(part 1 of 2)
# Autodesk Inventor assembly: SAR340
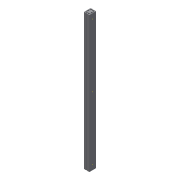
[picture p0: Inventor's stored thumbnail of the model, 180x180]
Saved by Autodesk Inventor 2020 (Build 240168000, 168)
## iProperties
Created: 2019-11-23
Part Number: SAR340
Catalog Web Link: www.cadenas.de
Description: SAR3-Slide Rails - Aluminum Alloy - Three-Step Slide Rails
Vendor: MISUMI
Document SubType Name: Assembly
Designer: psadmin
Manufacturer: MISUMI
Category: PARTsolutions
Company: MISUMI
PSOL_IDENT_0: {$CADENAS_DATA\23d-libs\misumi\metric\07_slide_rails\sar3_asmtab.prj},168 {VTYP=3D},{STYP=ASSTAB},{N
PSOL_IDENT_1: B=SAR340},{LINA=SAR340},{NN=SAR3},{DATE=09.09.2019 15:26:52},{GEOMDATE=01.03.2017 00:48:28},{VERSION=
PSOL_IDENT_2: },{LINEID=10},{WBVAR=NO},{WBNUMERIC=NO}  {NB=SAR340},{LINA=SAR340},{KT=DUMMY},{PN=SAR340},{TP=SAR3},
PSOL_IDENT_3: {TYPE=SAR3},{MAT1=Aluminum Alloy},{ST1=Clear Anodizing},{MAT2=Aluminum Alloy},{ST2=Clear Anodizing},
PSOL_IDENT_4: {MAT3=Steel},{NO=40},{RL=400},{TD=460},{A=185},{B=370},{C=185},{D=370},{RLO=147},{PPATH=sar3_series\
PSOL_IDENT_5: \sar3_templ.prj}
NN: SAR3
NT: Slide Rails - Aluminum Alloy - Three-Step Slide Rails
NB: SAR340
NBSYN: $PN.
LINA: SAR340
PN: SAR340
TP: SAR3
MAT1: Aluminum Alloy
ST1: Clear Anodizing
MAT2: Aluminum Alloy
ST2: Clear Anodizing
MAT3: Steel
NO: 40
RL: 400
TD: 460
A: 185
B: 370
C: 185
D: 370
RLO: 147
SUPPLIER: MISUMI
ARTICLENO: SAR340
BOMINFO: SAR340
CREATOR: CADENAS GmbH
Title: SAR340
Author: Cadenas PARTsolutions
Comments: Slide Rails - Aluminum Alloy - Three-Step Slide Rails
## Documents named in this file (4)
- C:\FTC\FTC8863CAD\Misumi\SAR340\SAR340.iam
- C:\FTC\FTC8863CAD\Misumi\SAR340\SAR340-40_r.ipt
- C:\FTC\FTC8863CAD\Misumi\SAR340\SAR340-40_b.ipt
- C:\FTC\FTC8863CAD\Misumi\SAR340\SAR3_ba.ipt
## Components (151 placed, 3 different names)
1. SAR340-40_r:1 — to_body_Z@1 <-> to_rail_Z@2, to_body_YZ@1 <-> to_rail_YZ@2, to_body2_Z@1 <-> to_rail_Z@3, to_body2_YZ@1 <-> to_rail_YZ@3, to_ball1_1_XY@1 <-> to_rail_XY@4, to_ball1_1_Z@1 <-> to_rail_Z@4, to_ball1_1_YZ@1 <-> to_rail_YZ@4, to_ball1_2_XY@1 <-> to_rail_XY@5, to_ball1_2_Z@1 <-> to_rail_Z@5, to_ball1_2_YZ@1 <-> to_rail_YZ@5, to_ball1_3_XY@1 <-> to_rail_XY@6, to_ball1_3_Z@1 <-> to_rail_Z@6, to_ball1_3_YZ@1 <-> to_rail_YZ@6, to_ball1_4_XY@1 <-> to_rail_XY@7, to_ball1_4_Z@1 <-> to_rail_Z@7, to_ball1_4_YZ@1 <-> to_rail_YZ@7, to_ball1_5_XY@1 <-> to_rail_XY@8, to_ball1_5_Z@1 <-> to_rail_Z@8, to_ball1_5_YZ@1 <-> to_rail_YZ@8, to_ball1_6_XY@1 <-> to_rail_XY@9, to_ball1_6_Z@1 <-> to_rail_Z@9, to_ball1_6_YZ@1 <-> to_rail_YZ@9, to_ball1_7_XY@1 <-> to_rail_XY@10, to_ball1_7_Z@1 <-> to_rail_Z@10, to_ball1_7_YZ@1 <-> to_rail_YZ@10, to_ball1_8_XY@1 <-> to_rail_XY@11, to_ball1_8_Z@1 <-> to_rail_Z@11, to_ball1_8_YZ@1 <-> to_rail_YZ@11, to_ball1_9_XY@1 <-> to_rail_XY@12, to_ball1_9_Z@1 <-> to_rail_Z@12, to_ball1_9_YZ@1 <-> to_rail_YZ@12, to_ball1_10_XY@1 <-> to_rail_XY@13, to_ball1_10_Z@1 <-> to_rail_Z@13, to_ball1_10_YZ@1 <-> to_rail_YZ@13, to_ball1_11_XY@1 <-> to_rail_XY@14, to_ball1_11_Z@1 <-> to_rail_Z@14, to_ball1_11_YZ@1 <-> to_rail_YZ@14, to_ball1_12_XY@1 <-> to_rail_XY@15, to_ball1_12_Z@1 <-> to_rail_Z@15, to_ball1_12_YZ@1 <-> to_rail_YZ@15, to_ball1_13_XY@1 <-> to_rail_XY@16, to_ball1_13_Z@1 <-> to_rail_Z@16, to_ball1_13_YZ@1 <-> to_rail_YZ@16, to_ball1_14_XY@1 <-> to_rail_XY@17, to_ball1_14_Z@1 <-> to_rail_Z@17, to_ball1_14_YZ@1 <-> to_rail_YZ@17, to_ball1_15_XY@1 <-> to_rail_XY@18, to_ball1_15_Z@1 <-> to_rail_Z@18, to_ball1_15_YZ@1 <-> to_rail_YZ@18, to_ball1_16_XY@1 <-> to_rail_XY@19, to_ball1_16_Z@1 <-> to_rail_Z@19, to_ball1_16_YZ@1 <-> to_rail_YZ@19, to_ball1_17_XY@1 <-> to_rail_XY@20, to_ball1_17_Z@1 <-> to_rail_Z@20, to_ball1_17_YZ@1 <-> to_rail_YZ@20, to_ball1_18_XY@1 <-> to_rail_XY@21, to_ball1_18_Z@1 <-> to_rail_Z@21, to_ball1_18_YZ@1 <-> to_rail_YZ@21, to_ball1_19_XY@1 <-> to_rail_XY@22, to_ball1_19_Z@1 <-> to_rail_Z@22, to_ball1_19_YZ@1 <-> to_rail_YZ@22, to_ball1_20_XY@1 <-> to_rail_XY@23, to_ball1_20_Z@1 <-> to_rail_Z@23, to_ball1_20_YZ@1 <-> to_rail_YZ@23, to_ball1_21_XY@1 <-> to_rail_XY@24, to_ball1_21_Z@1 <-> to_rail_Z@24, to_ball1_21_YZ@1 <-> to_rail_YZ@24, to_ball1_22_XY@1 <-> to_rail_XY@25, to_ball1_22_Z@1 <-> to_rail_Z@25, to_ball1_22_YZ@1 <-> to_rail_YZ@25, to_ball1_23_XY@1 <-> to_rail_XY@26, to_ball1_23_Z@1 <-> to_rail_Z@26, to_ball1_23_YZ@1 <-> to_rail_YZ@26, to_ball1_24_XY@1 <-> to_rail_XY@27, to_ball1_24_Z@1 <-> to_rail_Z@27, to_ball1_24_YZ@1 <-> to_rail_YZ@27, to_ball1_25_XY@1 <-> to_rail_XY@28, to_ball1_25_Z@1 <-> to_rail_Z@28, to_ball1_25_YZ@1 <-> to_rail_YZ@28, to_ball1_26_XY@1 <-> to_rail_XY@29, to_ball1_26_Z@1 <-> to_rail_Z@29, to_ball1_26_YZ@1 <-> to_rail_YZ@29, to_ball1_27_XY@1 <-> to_rail_XY@30, to_ball1_27_Z@1 <-> to_rail_Z@30, to_ball1_27_YZ@1 <-> to_rail_YZ@30, to_ball1_28_XY@1 <-> to_rail_XY@31, to_ball1_28_Z@1 <-> to_rail_Z@31, to_ball1_28_YZ@1 <-> to_rail_YZ@31, to_ball1_29_XY@1 <-> to_rail_XY@32, to_ball1_29_Z@1 <-> to_rail_Z@32, to_ball1_29_YZ@1 <-> to_rail_YZ@32, to_ball1_30_XY@1 <-> to_rail_XY@33, to_ball1_30_Z@1 <-> to_rail_Z@33, to_ball1_30_YZ@1 <-> to_rail_YZ@33, to_ball1_31_XY@1 <-> to_rail_XY@34, to_ball1_31_Z@1 <-> to_rail_Z@34, to_ball1_31_YZ@1 <-> to_rail_YZ@34, to_ball1_32_XY@1 <-> to_rail_XY@35, to_ball1_32_Z@1 <-> to_rail_Z@35, to_ball1_32_YZ@1 <-> to_rail_YZ@35, to_ball1_33_XY@1 <-> to_rail_XY@36, to_ball1_33_Z@1 <-> to_rail_Z@36, to_ball1_33_YZ@1 <-> to_rail_YZ@36, to_ball1_34_XY@1 <-> to_rail_XY@37, to_ball1_34_Z@1 <-> to_rail_Z@37, to_ball1_34_YZ@1 <-> to_rail_YZ@37, to_ball1_35_XY@1 <-> to_rail_XY@38, to_ball1_35_Z@1 <-> to_rail_Z@38, to_ball1_35_YZ@1 <-> to_rail_YZ@38, to_ball1_36_XY@1 <-> to_rail_XY@39, to_ball1_36_Z@1 <-> to_rail_Z@39, to_ball1_36_YZ@1 <-> to_rail_YZ@39, to_ball1_37_XY@1 <-> to_rail_XY@40, to_ball1_37_Z@1 <-> to_rail_Z@40, to_ball1_37_YZ@1 <-> to_rail_YZ@40, to_ball2_1_XY@1 <-> to_rail_XY@41, to_ball2_1_Z@1 <-> to_rail_Z@41, to_ball2_1_YZ@1 <-> to_rail_YZ@41, to_ball2_2_XY@1 <-> to_rail_XY@42, to_ball2_2_Z@1 <-> to_rail_Z@42, to_ball2_2_YZ@1 <-> to_rail_YZ@42, to_ball2_3_XY@1 <-> to_rail_XY@43, to_ball2_3_Z@1 <-> to_rail_Z@43, to_ball2_3_YZ@1 <-> to_rail_YZ@43, to_ball2_4_XY@1 <-> to_rail_XY@44, to_ball2_4_Z@1 <-> to_rail_Z@44, to_ball2_4_YZ@1 <-> to_rail_YZ@44, to_ball2_5_XY@1 <-> to_rail_XY@45, to_ball2_5_Z@1 <-> to_rail_Z@45, to_ball2_5_YZ@1 <-> to_rail_YZ@45, to_ball2_6_XY@1 <-> to_rail_XY@46, to_ball2_6_Z@1 <-> to_rail_Z@46, to_ball2_6_YZ@1 <-> to_rail_YZ@46, to_ball2_7_XY@1 <-> to_rail_XY@47, to_ball2_7_Z@1 <-> to_rail_Z@47, to_ball2_7_YZ@1 <-> to_rail_YZ@47, to_ball2_8_XY@1 <-> to_rail_XY@48, to_ball2_8_Z@1 <-> to_rail_Z@48, to_ball2_8_YZ@1 <-> to_rail_YZ@48, to_ball2_9_XY@1 <-> to_rail_XY@49, to_ball2_9_Z@1 <-> to_rail_Z@49, to_ball2_9_YZ@1 <-> to_rail_YZ@49, to_ball2_10_XY@1 <-> to_rail_XY@50, to_ball2_10_Z@1 <-> to_rail_Z@50, to_ball2_10_YZ@1 <-> to_rail_YZ@50, to_ball2_11_XY@1 <-> to_rail_XY@51, to_ball2_11_Z@1 <-> to_rail_Z@51, to_ball2_11_YZ@1 <-> to_rail_YZ@51, to_ball2_12_XY@1 <-> to_rail_XY@52, to_ball2_12_Z@1 <-> to_rail_Z@52, to_ball2_12_YZ@1 <-> to_rail_YZ@52, to_ball2_13_XY@1 <-> to_rail_XY@53, to_ball2_13_Z@1 <-> to_rail_Z@53, to_ball2_13_YZ@1 <-> to_rail_YZ@53, to_ball2_14_XY@1 <-> to_rail_XY@54, to_ball2_14_Z@1 <-> to_rail_Z@54, to_ball2_14_YZ@1 <-> to_rail_YZ@54, to_ball2_15_XY@1 <-> to_rail_XY@55, to_ball2_15_Z@1 <-> to_rail_Z@55, to_ball2_15_YZ@1 <-> to_rail_YZ@55, to_ball2_16_XY@1 <-> to_rail_XY@56, to_ball2_16_Z@1 <-> to_rail_Z@56, to_ball2_16_YZ@1 <-> to_rail_YZ@56, to_ball2_17_XY@1 <-> to_rail_XY@57, to_ball2_17_Z@1 <-> to_rail_Z@57, to_ball2_17_YZ@1 <-> to_rail_YZ@57, to_ball2_18_XY@1 <-> to_rail_XY@58, to_ball2_18_Z@1 <-> to_rail_Z@58, to_ball2_18_YZ@1 <-> to_rail_YZ@58, to_ball2_19_XY@1 <-> to_rail_XY@59, to_ball2_19_Z@1 <-> to_rail_Z@59, to_ball2_19_YZ@1 <-> to_rail_YZ@59, to_ball2_20_XY@1 <-> to_rail_XY@60, to_ball2_20_Z@1 <-> to_rail_Z@60, to_ball2_20_YZ@1 <-> to_rail_YZ@60, to_ball2_21_XY@1 <-> to_rail_XY@61, to_ball2_21_Z@1 <-> to_rail_Z@61, to_ball2_21_YZ@1 <-> to_rail_YZ@61, to_ball2_22_XY@1 <-> to_rail_XY@62, to_ball2_22_Z@1 <-> to_rail_Z@62, to_ball2_22_YZ@1 <-> to_rail_YZ@62, to_ball2_23_XY@1 <-> to_rail_XY@63, to_ball2_23_Z@1 <-> to_rail_Z@63, to_ball2_23_YZ@1 <-> to_rail_YZ@63, to_ball2_24_XY@1 <-> to_rail_XY@64, to_ball2_24_Z@1 <-> to_rail_Z@64, to_ball2_24_YZ@1 <-> to_rail_YZ@64, to_ball2_25_XY@1 <-> to_rail_XY@65, to_ball2_25_Z@1 <-> to_rail_Z@65, to_ball2_25_YZ@1 <-> to_rail_YZ@65, to_ball2_26_XY@1 <-> to_rail_XY@66, to_ball2_26_Z@1 <-> to_rail_Z@66, to_ball2_26_YZ@1 <-> to_rail_YZ@66, to_ball2_27_XY@1 <-> to_rail_XY@67, to_ball2_27_Z@1 <-> to_rail_Z@67, to_ball2_27_YZ@1 <-> to_rail_YZ@67, to_ball2_28_XY@1 <-> to_rail_XY@68, to_ball2_28_Z@1 <-> to_rail_Z@68, to_ball2_28_YZ@1 <-> to_rail_YZ@68, to_ball2_29_XY@1 <-> to_rail_XY@69, to_ball2_29_Z@1 <-> to_rail_Z@69, to_ball2_29_YZ@1 <-> to_rail_YZ@69, to_ball2_30_XY@1 <-> to_rail_XY@70, to_ball2_30_Z@1 <-> to_rail_Z@70, to_ball2_30_YZ@1 <-> to_rail_YZ@70, to_ball2_31_XY@1 <-> to_rail_XY@71, to_ball2_31_Z@1 <-> to_rail_Z@71, to_ball2_31_YZ@1 <-> to_rail_YZ@71, to_ball2_32_XY@1 <-> to_rail_XY@72, to_ball2_32_Z@1 <-> to_rail_Z@72, to_ball2_32_YZ@1 <-> to_rail_YZ@72, to_ball2_33_XY@1 <-> to_rail_XY@73, to_ball2_33_Z@1 <-> to_rail_Z@73, to_ball2_33_YZ@1 <-> to_rail_YZ@73, to_ball2_34_XY@1 <-> to_rail_XY@74, to_ball2_34_Z@1 <-> to_rail_Z@74, to_ball2_34_YZ@1 <-> to_rail_YZ@74, to_ball2_35_XY@1 <-> to_rail_XY@75, to_ball2_35_Z@1 <-> to_rail_Z@75, to_ball2_35_YZ@1 <-> to_rail_YZ@75, to_ball2_36_XY@1 <-> to_rail_XY@76, to_ball2_36_Z@1 <-> to_rail_Z@76, to_ball2_36_YZ@1 <-> to_rail_YZ@76, to_ball2_37_XY@1 <-> to_rail_XY@77, to_ball2_37_Z@1 <-> to_rail_Z@77, to_ball2_37_YZ@1 <-> to_rail_YZ@77, to_ball3_1_XY@1 <-> to_rail_XY@78, to_ball3_1_Z@1 <-> to_rail_Z@78, to_ball3_1_YZ@1 <-> to_rail_YZ@78, to_ball3_2_XY@1 <-> to_rail_XY@79, to_ball3_2_Z@1 <-> to_rail_Z@79, to_ball3_2_YZ@1 <-> to_rail_YZ@79, to_ball3_3_XY@1 <-> to_rail_XY@80, to_ball3_3_Z@1 <-> to_rail_Z@80, to_ball3_3_YZ@1 <-> to_rail_YZ@80, to_ball3_4_XY@1 <-> to_rail_XY@81, to_ball3_4_Z@1 <-> to_rail_Z@81, to_ball3_4_YZ@1 <-> to_rail_YZ@81, to_ball3_5_XY@1 <-> to_rail_XY@82, to_ball3_5_Z@1 <-> to_rail_Z@82, to_ball3_5_YZ@1 <-> to_rail_YZ@82, to_ball3_6_XY@1 <-> to_rail_XY@83, to_ball3_6_Z@1 <-> to_rail_Z@83, to_ball3_6_YZ@1 <-> to_rail_YZ@83, to_ball3_7_XY@1 <-> to_rail_XY@84, to_ball3_7_Z@1 <-> to_rail_Z@84, to_ball3_7_YZ@1 <-> to_rail_YZ@84, to_ball3_8_XY@1 <-> to_rail_XY@85, to_ball3_8_Z@1 <-> to_rail_Z@85, to_ball3_8_YZ@1 <-> to_rail_YZ@85, to_ball3_9_XY@1 <-> to_rail_XY@86, to_ball3_9_Z@1 <-> to_rail_Z@86, to_ball3_9_YZ@1 <-> to_rail_YZ@86, to_ball3_10_XY@1 <-> to_rail_XY@87, to_ball3_10_Z@1 <-> to_rail_Z@87, to_ball3_10_YZ@1 <-> to_rail_YZ@87, to_ball3_11_XY@1 <-> to_rail_XY@88, to_ball3_11_Z@1 <-> to_rail_Z@88, to_ball3_11_YZ@1 <-> to_rail_YZ@88, to_ball3_12_XY@1 <-> to_rail_XY@89, to_ball3_12_Z@1 <-> to_rail_Z@89, to_ball3_12_YZ@1 <-> to_rail_YZ@89, to_ball3_13_XY@1 <-> to_rail_XY@90, to_ball3_13_Z@1 <-> to_rail_Z@90, to_ball3_13_YZ@1 <-> to_rail_YZ@90, to_ball3_14_XY@1 <-> to_rail_XY@91, to_ball3_14_Z@1 <-> to_rail_Z@91, to_ball3_14_YZ@1 <-> to_rail_YZ@91, to_ball3_15_XY@1 <-> to_rail_XY@92, to_ball3_15_Z@1 <-> to_rail_Z@92, to_ball3_15_YZ@1 <-> to_rail_YZ@92, to_ball3_16_XY@1 <-> to_rail_XY@93, to_ball3_16_Z@1 <-> to_rail_Z@93, to_ball3_16_YZ@1 <-> to_rail_YZ@93, to_ball3_17_XY@1 <-> to_rail_XY@94, to_ball3_17_Z@1 <-> to_rail_Z@94, to_ball3_17_YZ@1 <-> to_rail_YZ@94, to_ball3_18_XY@1 <-> to_rail_XY@95, to_ball3_18_Z@1 <-> to_rail_Z@95, to_ball3_18_YZ@1 <-> to_rail_YZ@95, to_ball3_19_XY@1 <-> to_rail_XY@96, to_ball3_19_Z@1 <-> to_rail_Z@96, to_ball3_19_YZ@1 <-> to_rail_YZ@96, to_ball3_20_XY@1 <-> to_rail_XY@97, to_ball3_20_Z@1 <-> to_rail_Z@97, to_ball3_20_YZ@1 <-> to_rail_YZ@97, to_ball3_21_XY@1 <-> to_rail_XY@98, to_ball3_21_Z@1 <-> to_rail_Z@98, to_ball3_21_YZ@1 <-> to_rail_YZ@98, to_ball3_22_XY@1 <-> to_rail_XY@99, to_ball3_22_Z@1 <-> to_rail_Z@99, to_ball3_22_YZ@1 <-> to_rail_YZ@99, to_ball3_23_XY@1 <-> to_rail_XY@100, to_ball3_23_Z@1 <-> to_rail_Z@100, to_ball3_23_YZ@1 <-> to_rail_YZ@100, to_ball3_24_XY@1 <-> to_rail_XY@101, to_ball3_24_Z@1 <-> to_rail_Z@101, to_ball3_24_YZ@1 <-> to_rail_YZ@101, to_ball3_25_XY@1 <-> to_rail_XY@102, to_ball3_25_Z@1 <-> to_rail_Z@102, to_ball3_25_YZ@1 <-> to_rail_YZ@102, to_ball3_26_XY@1 <-> to_rail_XY@103, to_ball3_26_Z@1 <-> to_rail_Z@103, to_ball3_26_YZ@1 <-> to_rail_YZ@103, to_ball3_27_XY@1 <-> to_rail_XY@104, to_ball3_27_Z@1 <-> to_rail_Z@104, to_ball3_27_YZ@1 <-> to_rail_YZ@104, to_ball3_28_XY@1 <-> to_rail_XY@105, to_ball3_28_Z@1 <-> to_rail_Z@105, to_ball3_28_YZ@1 <-> to_rail_YZ@105, to_ball3_29_XY@1 <-> to_rail_XY@106, to_ball3_29_Z@1 <-> to_rail_Z@106, to_ball3_29_YZ@1 <-> to_rail_YZ@106, to_ball3_30_XY@1 <-> to_rail_XY@107, to_ball3_30_Z@1 <-> to_rail_Z@107, to_ball3_30_YZ@1 <-> to_rail_YZ@107, to_ball3_31_XY@1 <-> to_rail_XY@108, to_ball3_31_Z@1 <-> to_rail_Z@108, to_ball3_31_YZ@1 <-> to_rail_YZ@108, to_ball3_32_XY@1 <-> to_rail_XY@109, to_ball3_32_Z@1 <-> to_rail_Z@109, to_ball3_32_YZ@1 <-> to_rail_YZ@109, to_ball3_33_XY@1 <-> to_rail_XY@110, to_ball3_33_Z@1 <-> to_rail_Z@110, to_ball3_33_YZ@1 <-> to_rail_YZ@110, to_ball3_34_XY@1 <-> to_rail_XY@111, to_ball3_34_Z@1 <-> to_rail_Z@111, to_ball3_34_YZ@1 <-> to_rail_YZ@111, to_ball3_35_XY@1 <-> to_rail_XY@112, to_ball3_35_Z@1 <-> to_rail_Z@112, to_ball3_35_YZ@1 <-> to_rail_YZ@112, to_ball3_36_XY@1 <-> to_rail_XY@113, to_ball3_36_Z@1 <-> to_rail_Z@113, to_ball3_36_YZ@1 <-> to_rail_YZ@113, to_ball3_37_XY@1 <-> to_rail_XY@114, to_ball3_37_Z@1 <-> to_rail_Z@114, to_ball3_37_YZ@1 <-> to_rail_YZ@114, to_ball4_1_XY@1 <-> to_rail_XY@115, to_ball4_1_Z@1 <-> to_rail_Z@115, to_ball4_1_YZ@1 <-> to_rail_YZ@115, to_ball4_2_XY@1 <-> to_rail_XY@116, to_ball4_2_Z@1 <-> to_rail_Z@116, to_ball4_2_YZ@1 <-> to_rail_YZ@116, to_ball4_3_XY@1 <-> to_rail_XY@117, to_ball4_3_Z@1 <-> to_rail_Z@117, to_ball4_3_YZ@1 <-> to_rail_YZ@117, to_ball4_4_XY@1 <-> to_rail_XY@118, to_ball4_4_Z@1 <-> to_rail_Z@118, to_ball4_4_YZ@1 <-> to_rail_YZ@118, to_ball4_5_XY@1 <-> to_rail_XY@119, to_ball4_5_Z@1 <-> to_rail_Z@119, to_ball4_5_YZ@1 <-> to_rail_YZ@119, to_ball4_6_XY@1 <-> to_rail_XY@120, to_ball4_6_Z@1 <-> to_rail_Z@120, to_ball4_6_YZ@1 <-> to_rail_YZ@120, to_ball4_7_XY@1 <-> to_rail_XY@121, to_ball4_7_Z@1 <-> to_rail_Z@121, to_ball4_7_YZ@1 <-> to_rail_YZ@121, to_ball4_8_XY@1 <-> to_rail_XY@122, to_ball4_8_Z@1 <-> to_rail_Z@122, to_ball4_8_YZ@1 <-> to_rail_YZ@122, to_ball4_9_XY@1 <-> to_rail_XY@123, to_ball4_9_Z@1 <-> to_rail_Z@123, to_ball4_9_YZ@1 <-> to_rail_YZ@123, to_ball4_10_XY@1 <-> to_rail_XY@124, to_ball4_10_Z@1 <-> to_rail_Z@124, to_ball4_10_YZ@1 <-> to_rail_YZ@124, to_ball4_11_XY@1 <-> to_rail_XY@125, to_ball4_11_Z@1 <-> to_rail_Z@125, to_ball4_11_YZ@1 <-> to_rail_YZ@125, to_ball4_12_XY@1 <-> to_rail_XY@126, to_ball4_12_Z@1 <-> to_rail_Z@126, to_ball4_12_YZ@1 <-> to_rail_YZ@126, to_ball4_13_XY@1 <-> to_rail_XY@127, to_ball4_13_Z@1 <-> to_rail_Z@127, to_ball4_13_YZ@1 <-> to_rail_YZ@127, to_ball4_14_XY@1 <-> to_rail_XY@128, to_ball4_14_Z@1 <-> to_rail_Z@128, to_ball4_14_YZ@1 <-> to_rail_YZ@128, to_ball4_15_XY@1 <-> to_rail_XY@129, to_ball4_15_Z@1 <-> to_rail_Z@129, to_ball4_15_YZ@1 <-> to_rail_YZ@129, to_ball4_16_XY@1 <-> to_rail_XY@130, to_ball4_16_Z@1 <-> to_rail_Z@130, to_ball4_16_YZ@1 <-> to_rail_YZ@130, to_ball4_17_XY@1 <-> to_rail_XY@131, to_ball4_17_Z@1 <-> to_rail_Z@131, to_ball4_17_YZ@1 <-> to_rail_YZ@131, to_ball4_18_XY@1 <-> to_rail_XY@132, to_ball4_18_Z@1 <-> to_rail_Z@132, to_ball4_18_YZ@1 <-> to_rail_YZ@132, to_ball4_19_XY@1 <-> to_rail_XY@133, to_ball4_19_Z@1 <-> to_rail_Z@133, to_ball4_19_YZ@1 <-> to_rail_YZ@133, to_ball4_20_XY@1 <-> to_rail_XY@134, to_ball4_20_Z@1 <-> to_rail_Z@134, to_ball4_20_YZ@1 <-> to_rail_YZ@134, to_ball4_21_XY@1 <-> to_rail_XY@135, to_ball4_21_Z@1 <-> to_rail_Z@135, to_ball4_21_YZ@1 <-> to_rail_YZ@135, to_ball4_22_XY@1 <-> to_rail_XY@136, to_ball4_22_Z@1 <-> to_rail_Z@136, to_ball4_22_YZ@1 <-> to_rail_YZ@136, to_ball4_23_XY@1 <-> to_rail_XY@137, to_ball4_23_Z@1 <-> to_rail_Z@137, to_ball4_23_YZ@1 <-> to_rail_YZ@137, to_ball4_24_XY@1 <-> to_rail_XY@138, to_ball4_24_Z@1 <-> to_rail_Z@138, to_ball4_24_YZ@1 <-> to_rail_YZ@138, to_ball4_25_XY@1 <-> to_rail_XY@139, to_ball4_25_Z@1 <-> to_rail_Z@139, to_ball4_25_YZ@1 <-> to_rail_YZ@139, to_ball4_26_XY@1 <-> to_rail_XY@140, to_ball4_26_Z@1 <-> to_rail_Z@140, to_ball4_26_YZ@1 <-> to_rail_YZ@140, to_ball4_27_XY@1 <-> to_rail_XY@141, to_ball4_27_Z@1 <-> to_rail_Z@141, to_ball4_27_YZ@1 <-> to_rail_YZ@141, to_ball4_28_XY@1 <-> to_rail_XY@142, to_ball4_28_Z@1 <-> to_rail_Z@142, to_ball4_28_YZ@1 <-> to_rail_YZ@142, to_ball4_29_XY@1 <-> to_rail_XY@143, to_ball4_29_Z@1 <-> to_rail_Z@143, to_ball4_29_YZ@1 <-> to_rail_YZ@143, to_ball4_30_XY@1 <-> to_rail_XY@144, to_ball4_30_Z@1 <-> to_rail_Z@144, to_ball4_30_YZ@1 <-> to_rail_YZ@144, to_ball4_31_XY@1 <-> to_rail_XY@145, to_ball4_31_Z@1 <-> to_rail_Z@145, to_ball4_31_YZ@1 <-> to_rail_YZ@145, to_ball4_32_XY@1 <-> to_rail_XY@146, to_ball4_32_Z@1 <-> to_rail_Z@146, to_ball4_32_YZ@1 <-> to_rail_YZ@146, to_ball4_33_XY@1 <-> to_rail_XY@147, to_ball4_33_Z@1 <-> to_rail_Z@147, to_ball4_33_YZ@1 <-> to_rail_YZ@147, to_ball4_34_XY@1 <-> to_rail_XY@148, to_ball4_34_Z@1 <-> to_rail_Z@148, to_ball4_34_YZ@1 <-> to_rail_YZ@148, to_ball4_35_XY@1 <-> to_rail_XY@149, to_ball4_35_Z@1 <-> to_rail_Z@149, to_ball4_35_YZ@1 <-> to_rail_YZ@149, to_ball4_36_XY@1 <-> to_rail_XY@150, to_ball4_36_Z@1 <-> to_rail_Z@150, to_ball4_36_YZ@1 <-> to_rail_YZ@150, to_ball4_37_XY@1 <-> to_rail_XY@151, to_ball4_37_Z@1 <-> to_rail_Z@151, to_ball4_37_YZ@1 <-> to_rail_YZ@151
2. SAR340-40_b:1 — to_body_Z@1 <-> to_rail_Z@2, to_body_YZ@1 <-> to_rail_YZ@2, Mate:302, Mate:303, Mate:304
3. SAR340-40_b:2 — to_body2_Z@1 <-> to_rail_Z@3, to_body2_YZ@1 <-> to_rail_YZ@3, Mate:299, Mate:300, Mate:301
4. SAR3_ba:1 — to_ball1_1_XY@1 <-> to_rail_XY@4, to_ball1_1_Z@1 <-> to_rail_Z@4, to_ball1_1_YZ@1 <-> to_rail_YZ@4
5. SAR3_ba:2 — to_ball1_2_XY@1 <-> to_rail_XY@5, to_ball1_2_Z@1 <-> to_rail_Z@5, to_ball1_2_YZ@1 <-> to_rail_YZ@5
6. SAR3_ba:3 — to_ball1_3_XY@1 <-> to_rail_XY@6, to_ball1_3_Z@1 <-> to_rail_Z@6, to_ball1_3_YZ@1 <-> to_rail_YZ@6
7. SAR3_ba:4 — to_ball1_4_XY@1 <-> to_rail_XY@7, to_ball1_4_Z@1 <-> to_rail_Z@7, to_ball1_4_YZ@1 <-> to_rail_YZ@7
8. SAR3_ba:5 — to_ball1_5_XY@1 <-> to_rail_XY@8, to_ball1_5_Z@1 <-> to_rail_Z@8, to_ball1_5_YZ@1 <-> to_rail_YZ@8
9. SAR3_ba:6 — to_ball1_6_XY@1 <-> to_rail_XY@9, to_ball1_6_Z@1 <-> to_rail_Z@9, to_ball1_6_YZ@1 <-> to_rail_YZ@9
10. SAR3_ba:7 — to_ball1_7_XY@1 <-> to_rail_XY@10, to_ball1_7_Z@1 <-> to_rail_Z@10, to_ball1_7_YZ@1 <-> to_rail_YZ@10
11. SAR3_ba:8 — to_ball1_8_XY@1 <-> to_rail_XY@11, to_ball1_8_Z@1 <-> to_rail_Z@11, to_ball1_8_YZ@1 <-> to_rail_YZ@11
12. SAR3_ba:9 — to_ball1_9_XY@1 <-> to_rail_XY@12, to_ball1_9_Z@1 <-> to_rail_Z@12, to_ball1_9_YZ@1 <-> to_rail_YZ@12
13. SAR3_ba:10 — to_ball1_10_XY@1 <-> to_rail_XY@13, to_ball1_10_Z@1 <-> to_rail_Z@13, to_ball1_10_YZ@1 <-> to_rail_YZ@13
14. SAR3_ba:11 — to_ball1_11_XY@1 <-> to_rail_XY@14, to_ball1_11_Z@1 <-> to_rail_Z@14, to_ball1_11_YZ@1 <-> to_rail_YZ@14
15. SAR3_ba:12 — to_ball1_12_XY@1 <-> to_rail_XY@15, to_ball1_12_Z@1 <-> to_rail_Z@15, to_ball1_12_YZ@1 <-> to_rail_YZ@15
16. SAR3_ba:13 — to_ball1_13_XY@1 <-> to_rail_XY@16, to_ball1_13_Z@1 <-> to_rail_Z@16, to_ball1_13_YZ@1 <-> to_rail_YZ@16
17. SAR3_ba:14 — to_ball1_14_XY@1 <-> to_rail_XY@17, to_ball1_14_Z@1 <-> to_rail_Z@17, to_ball1_14_YZ@1 <-> to_rail_YZ@17
18. SAR3_ba:15 — to_ball1_15_XY@1 <-> to_rail_XY@18, to_ball1_15_Z@1 <-> to_rail_Z@18, to_ball1_15_YZ@1 <-> to_rail_YZ@18
19. SAR3_ba:16 — to_ball1_16_XY@1 <-> to_rail_XY@19, to_ball1_16_Z@1 <-> to_rail_Z@19, to_ball1_16_YZ@1 <-> to_rail_YZ@19
20. SAR3_ba:17 — to_ball1_17_XY@1 <-> to_rail_XY@20, to_ball1_17_Z@1 <-> to_rail_Z@20, to_ball1_17_YZ@1 <-> to_rail_YZ@20
21. SAR3_ba:18 — to_ball1_18_XY@1 <-> to_rail_XY@21, to_ball1_18_Z@1 <-> to_rail_Z@21, to_ball1_18_YZ@1 <-> to_rail_YZ@21
22. SAR3_ba:19 — to_ball1_19_XY@1 <-> to_rail_XY@22, to_ball1_19_Z@1 <-> to_rail_Z@22, to_ball1_19_YZ@1 <-> to_rail_YZ@22
23. SAR3_ba:20 — to_ball1_20_XY@1 <-> to_rail_XY@23, to_ball1_20_Z@1 <-> to_rail_Z@23, to_ball1_20_YZ@1 <-> to_rail_YZ@23
24. SAR3_ba:21 — to_ball1_21_XY@1 <-> to_rail_XY@24, to_ball1_21_Z@1 <-> to_rail_Z@24, to_ball1_21_YZ@1 <-> to_rail_YZ@24
25. SAR3_ba:22 — to_ball1_22_XY@1 <-> to_rail_XY@25, to_ball1_22_Z@1 <-> to_rail_Z@25, to_ball1_22_YZ@1 <-> to_rail_YZ@25
26. SAR3_ba:23 — to_ball1_23_XY@1 <-> to_rail_XY@26, to_ball1_23_Z@1 <-> to_rail_Z@26, to_ball1_23_YZ@1 <-> to_rail_YZ@26
27. SAR3_ba:24 — to_ball1_24_XY@1 <-> to_rail_XY@27, to_ball1_24_Z@1 <-> to_rail_Z@27, to_ball1_24_YZ@1 <-> to_rail_YZ@27
28. SAR3_ba:25 — to_ball1_25_XY@1 <-> to_rail_XY@28, to_ball1_25_Z@1 <-> to_rail_Z@28, to_ball1_25_YZ@1 <-> to_rail_YZ@28
29. SAR3_ba:26 — to_ball1_26_XY@1 <-> to_rail_XY@29, to_ball1_26_Z@1 <-> to_rail_Z@29, to_ball1_26_YZ@1 <-> to_rail_YZ@29
30. SAR3_ba:27 — to_ball1_27_XY@1 <-> to_rail_XY@30, to_ball1_27_Z@1 <-> to_rail_Z@30, to_ball1_27_YZ@1 <-> to_rail_YZ@30
31. SAR3_ba:28 — to_ball1_28_XY@1 <-> to_rail_XY@31, to_ball1_28_Z@1 <-> to_rail_Z@31, to_ball1_28_YZ@1 <-> to_rail_YZ@31
32. SAR3_ba:29 — to_ball1_29_XY@1 <-> to_rail_XY@32, to_ball1_29_Z@1 <-> to_rail_Z@32, to_ball1_29_YZ@1 <-> to_rail_YZ@32
33. SAR3_ba:30 — to_ball1_30_XY@1 <-> to_rail_XY@33, to_ball1_30_Z@1 <-> to_rail_Z@33, to_ball1_30_YZ@1 <-> to_rail_YZ@33
34. SAR3_ba:31 — to_ball1_31_XY@1 <-> to_rail_XY@34, to_ball1_31_Z@1 <-> to_rail_Z@34, to_ball1_31_YZ@1 <-> to_rail_YZ@34
35. SAR3_ba:32 — to_ball1_32_XY@1 <-> to_rail_XY@35, to_ball1_32_Z@1 <-> to_rail_Z@35, to_ball1_32_YZ@1 <-> to_rail_YZ@35
36. SAR3_ba:33 — to_ball1_33_XY@1 <-> to_rail_XY@36, to_ball1_33_Z@1 <-> to_rail_Z@36, to_ball1_33_YZ@1 <-> to_rail_YZ@36
37. SAR3_ba:34 — to_ball1_34_XY@1 <-> to_rail_XY@37, to_ball1_34_Z@1 <-> to_rail_Z@37, to_ball1_34_YZ@1 <-> to_rail_YZ@37
38. SAR3_ba:35 — to_ball1_35_XY@1 <-> to_rail_XY@38, to_ball1_35_Z@1 <-> to_rail_Z@38, to_ball1_35_YZ@1 <-> to_rail_YZ@38
39. SAR3_ba:36 — to_ball1_36_XY@1 <-> to_rail_XY@39, to_ball1_36_Z@1 <-> to_rail_Z@39, to_ball1_36_YZ@1 <-> to_rail_YZ@39
40. SAR3_ba:37 — to_ball1_37_XY@1 <-> to_rail_XY@40, to_ball1_37_Z@1 <-> to_rail_Z@40, to_ball1_37_YZ@1 <-> to_rail_YZ@40
41. SAR3_ba:38 — to_ball2_1_XY@1 <-> to_rail_XY@41, to_ball2_1_Z@1 <-> to_rail_Z@41, to_ball2_1_YZ@1 <-> to_rail_YZ@41
42. SAR3_ba:39 — to_ball2_2_XY@1 <-> to_rail_XY@42, to_ball2_2_Z@1 <-> to_rail_Z@42, to_ball2_2_YZ@1 <-> to_rail_YZ@42
43. SAR3_ba:40 — to_ball2_3_XY@1 <-> to_rail_XY@43, to_ball2_3_Z@1 <-> to_rail_Z@43, to_ball2_3_YZ@1 <-> to_rail_YZ@43
44. SAR3_ba:41 — to_ball2_4_XY@1 <-> to_rail_XY@44, to_ball2_4_Z@1 <-> to_rail_Z@44, to_ball2_4_YZ@1 <-> to_rail_YZ@44
45. SAR3_ba:42 — to_ball2_5_XY@1 <-> to_rail_XY@45, to_ball2_5_Z@1 <-> to_rail_Z@45, to_ball2_5_YZ@1 <-> to_rail_YZ@45
46. SAR3_ba:43 — to_ball2_6_XY@1 <-> to_rail_XY@46, to_ball2_6_Z@1 <-> to_rail_Z@46, to_ball2_6_YZ@1 <-> to_rail_YZ@46
47. SAR3_ba:44 — to_ball2_7_XY@1 <-> to_rail_XY@47, to_ball2_7_Z@1 <-> to_rail_Z@47, to_ball2_7_YZ@1 <-> to_rail_YZ@47
48. SAR3_ba:45 — to_ball2_8_XY@1 <-> to_rail_XY@48, to_ball2_8_Z@1 <-> to_rail_Z@48, to_ball2_8_YZ@1 <-> to_rail_YZ@48
49. SAR3_ba:46 — to_ball2_9_XY@1 <-> to_rail_XY@49, to_ball2_9_Z@1 <-> to_rail_Z@49, to_ball2_9_YZ@1 <-> to_rail_YZ@49
50. SAR3_ba:47 — to_ball2_10_XY@1 <-> to_rail_XY@50, to_ball2_10_Z@1 <-> to_rail_Z@50, to_ball2_10_YZ@1 <-> to_rail_YZ@50
51. SAR3_ba:48 — to_ball2_11_XY@1 <-> to_rail_XY@51, to_ball2_11_Z@1 <-> to_rail_Z@51, to_ball2_11_YZ@1 <-> to_rail_YZ@51
52. SAR3_ba:49 — to_ball2_12_XY@1 <-> to_rail_XY@52, to_ball2_12_Z@1 <-> to_rail_Z@52, to_ball2_12_YZ@1 <-> to_rail_YZ@52
53. SAR3_ba:50 — to_ball2_13_XY@1 <-> to_rail_XY@53, to_ball2_13_Z@1 <-> to_rail_Z@53, to_ball2_13_YZ@1 <-> to_rail_YZ@53
54. SAR3_ba:51 — to_ball2_14_XY@1 <-> to_rail_XY@54, to_ball2_14_Z@1 <-> to_rail_Z@54, to_ball2_14_YZ@1 <-> to_rail_YZ@54
55. SAR3_ba:52 — to_ball2_15_XY@1 <-> to_rail_XY@55, to_ball2_15_Z@1 <-> to_rail_Z@55, to_ball2_15_YZ@1 <-> to_rail_YZ@55
56. SAR3_ba:53 — to_ball2_16_XY@1 <-> to_rail_XY@56, to_ball2_16_Z@1 <-> to_rail_Z@56, to_ball2_16_YZ@1 <-> to_rail_YZ@56
57. SAR3_ba:54 — to_ball2_17_XY@1 <-> to_rail_XY@57, to_ball2_17_Z@1 <-> to_rail_Z@57, to_ball2_17_YZ@1 <-> to_rail_YZ@57
58. SAR3_ba:55 — to_ball2_18_XY@1 <-> to_rail_XY@58, to_ball2_18_Z@1 <-> to_rail_Z@58, to_ball2_18_YZ@1 <-> to_rail_YZ@58
59. SAR3_ba:56 — to_ball2_19_XY@1 <-> to_rail_XY@59, to_ball2_19_Z@1 <-> to_rail_Z@59, to_ball2_19_YZ@1 <-> to_rail_YZ@59
60. SAR3_ba:57 — to_ball2_20_XY@1 <-> to_rail_XY@60, to_ball2_20_Z@1 <-> to_rail_Z@60, to_ball2_20_YZ@1 <-> to_rail_YZ@60
61. SAR3_ba:58 — to_ball2_21_XY@1 <-> to_rail_XY@61, to_ball2_21_Z@1 <-> to_rail_Z@61, to_ball2_21_YZ@1 <-> to_rail_YZ@61
62. SAR3_ba:59 — to_ball2_22_XY@1 <-> to_rail_XY@62, to_ball2_22_Z@1 <-> to_rail_Z@62, to_ball2_22_YZ@1 <-> to_rail_YZ@62
63. SAR3_ba:60 — to_ball2_23_XY@1 <-> to_rail_XY@63, to_ball2_23_Z@1 <-> to_rail_Z@63, to_ball2_23_YZ@1 <-> to_rail_YZ@63
64. SAR3_ba:61 — to_ball2_24_XY@1 <-> to_rail_XY@64, to_ball2_24_Z@1 <-> to_rail_Z@64, to_ball2_24_YZ@1 <-> to_rail_YZ@64
65. SAR3_ba:62 — to_ball2_25_XY@1 <-> to_rail_XY@65, to_ball2_25_Z@1 <-> to_rail_Z@65, to_ball2_25_YZ@1 <-> to_rail_YZ@65
66. SAR3_ba:63 — to_ball2_26_XY@1 <-> to_rail_XY@66, to_ball2_26_Z@1 <-> to_rail_Z@66, to_ball2_26_YZ@1 <-> to_rail_YZ@66
67. SAR3_ba:64 — to_ball2_27_XY@1 <-> to_rail_XY@67, to_ball2_27_Z@1 <-> to_rail_Z@67, to_ball2_27_YZ@1 <-> to_rail_YZ@67
68. SAR3_ba:65 — to_ball2_28_XY@1 <-> to_rail_XY@68, to_ball2_28_Z@1 <-> to_rail_Z@68, to_ball2_28_YZ@1 <-> to_rail_YZ@68
69. SAR3_ba:66 — to_ball2_29_XY@1 <-> to_rail_XY@69, to_ball2_29_Z@1 <-> to_rail_Z@69, to_ball2_29_YZ@1 <-> to_rail_YZ@69
70. SAR3_ba:67 — to_ball2_30_XY@1 <-> to_rail_XY@70, to_ball2_30_Z@1 <-> to_rail_Z@70, to_ball2_30_YZ@1 <-> to_rail_YZ@70
71. SAR3_ba:68 — to_ball2_31_XY@1 <-> to_rail_XY@71, to_ball2_31_Z@1 <-> to_rail_Z@71, to_ball2_31_YZ@1 <-> to_rail_YZ@71
72. SAR3_ba:69 — to_ball2_32_XY@1 <-> to_rail_XY@72, to_ball2_32_Z@1 <-> to_rail_Z@72, to_ball2_32_YZ@1 <-> to_rail_YZ@72
73. SAR3_ba:70 — to_ball2_33_XY@1 <-> to_rail_XY@73, to_ball2_33_Z@1 <-> to_rail_Z@73, to_ball2_33_YZ@1 <-> to_rail_YZ@73
74. SAR3_ba:71 — to_ball2_34_XY@1 <-> to_rail_XY@74, to_ball2_34_Z@1 <-> to_rail_Z@74, to_ball2_34_YZ@1 <-> to_rail_YZ@74
75. SAR3_ba:72 — to_ball2_35_XY@1 <-> to_rail_XY@75, to_ball2_35_Z@1 <-> to_rail_Z@75, to_ball2_35_YZ@1 <-> to_rail_YZ@75
76. SAR3_ba:73 — to_ball2_36_XY@1 <-> to_rail_XY@76, to_ball2_36_Z@1 <-> to_rail_Z@76, to_ball2_36_YZ@1 <-> to_rail_YZ@76
77. SAR3_ba:74 — to_ball2_37_XY@1 <-> to_rail_XY@77, to_ball2_37_Z@1 <-> to_rail_Z@77, to_ball2_37_YZ@1 <-> to_rail_YZ@77
78. SAR3_ba:75 — to_ball3_1_XY@1 <-> to_rail_XY@78, to_ball3_1_Z@1 <-> to_rail_Z@78, to_ball3_1_YZ@1 <-> to_rail_YZ@78
79. SAR3_ba:76 — to_ball3_2_XY@1 <-> to_rail_XY@79, to_ball3_2_Z@1 <-> to_rail_Z@79, to_ball3_2_YZ@1 <-> to_rail_YZ@79
80. SAR3_ba:77 — to_ball3_3_XY@1 <-> to_rail_XY@80, to_ball3_3_Z@1 <-> to_rail_Z@80, to_ball3_3_YZ@1 <-> to_rail_YZ@80
81. SAR3_ba:78 — to_ball3_4_XY@1 <-> to_rail_XY@81, to_ball3_4_Z@1 <-> to_rail_Z@81, to_ball3_4_YZ@1 <-> to_rail_YZ@81
82. SAR3_ba:79 — to_ball3_5_XY@1 <-> to_rail_XY@82, to_ball3_5_Z@1 <-> to_rail_Z@82, to_ball3_5_YZ@1 <-> to_rail_YZ@82
83. SAR3_ba:80 — to_ball3_6_XY@1 <-> to_rail_XY@83, to_ball3_6_Z@1 <-> to_rail_Z@83, to_ball3_6_YZ@1 <-> to_rail_YZ@83
84. SAR3_ba:81 — to_ball3_7_XY@1 <-> to_rail_XY@84, to_ball3_7_Z@1 <-> to_rail_Z@84, to_ball3_7_YZ@1 <-> to_rail_YZ@84
85. SAR3_ba:82 — to_ball3_8_XY@1 <-> to_rail_XY@85, to_ball3_8_Z@1 <-> to_rail_Z@85, to_ball3_8_YZ@1 <-> to_rail_YZ@85
86. SAR3_ba:83 — to_ball3_9_XY@1 <-> to_rail_XY@86, to_ball3_9_Z@1 <-> to_rail_Z@86, to_ball3_9_YZ@1 <-> to_rail_YZ@86
87. SAR3_ba:84 — to_ball3_10_XY@1 <-> to_rail_XY@87, to_ball3_10_Z@1 <-> to_rail_Z@87, to_ball3_10_YZ@1 <-> to_rail_YZ@87
88. SAR3_ba:85 — to_ball3_11_XY@1 <-> to_rail_XY@88, to_ball3_11_Z@1 <-> to_rail_Z@88, to_ball3_11_YZ@1 <-> to_rail_YZ@88
89. SAR3_ba:86 — to_ball3_12_XY@1 <-> to_rail_XY@89, to_ball3_12_Z@1 <-> to_rail_Z@89, to_ball3_12_YZ@1 <-> to_rail_YZ@89
90. SAR3_ba:87 — to_ball3_13_XY@1 <-> to_rail_XY@90, to_ball3_13_Z@1 <-> to_rail_Z@90, to_ball3_13_YZ@1 <-> to_rail_YZ@90
91. SAR3_ba:88 — to_ball3_14_XY@1 <-> to_rail_XY@91, to_ball3_14_Z@1 <-> to_rail_Z@91, to_ball3_14_YZ@1 <-> to_rail_YZ@91
92. SAR3_ba:89 — to_ball3_15_XY@1 <-> to_rail_XY@92, to_ball3_15_Z@1 <-> to_rail_Z@92, to_ball3_15_YZ@1 <-> to_rail_YZ@92
93. SAR3_ba:90 — to_ball3_16_XY@1 <-> to_rail_XY@93, to_ball3_16_Z@1 <-> to_rail_Z@93, to_ball3_16_YZ@1 <-> to_rail_YZ@93
94. SAR3_ba:91 — to_ball3_17_XY@1 <-> to_rail_XY@94, to_ball3_17_Z@1 <-> to_rail_Z@94, to_ball3_17_YZ@1 <-> to_rail_YZ@94
95. SAR3_ba:92 — to_ball3_18_XY@1 <-> to_rail_XY@95, to_ball3_18_Z@1 <-> to_rail_Z@95, to_ball3_18_YZ@1 <-> to_rail_YZ@95
96. SAR3_ba:93 — to_ball3_19_XY@1 <-> to_rail_XY@96, to_ball3_19_Z@1 <-> to_rail_Z@96, to_ball3_19_YZ@1 <-> to_rail_YZ@96
97. SAR3_ba:94 — to_ball3_20_XY@1 <-> to_rail_XY@97, to_ball3_20_Z@1 <-> to_rail_Z@97, to_ball3_20_YZ@1 <-> to_rail_YZ@97
98. SAR3_ba:95 — to_ball3_21_XY@1 <-> to_rail_XY@98, to_ball3_21_Z@1 <-> to_rail_Z@98, to_ball3_21_YZ@1 <-> to_rail_YZ@98
99. SAR3_ba:96 — to_ball3_22_XY@1 <-> to_rail_XY@99, to_ball3_22_Z@1 <-> to_rail_Z@99, to_ball3_22_YZ@1 <-> to_rail_YZ@99
100. SAR3_ba:97 — to_ball3_23_XY@1 <-> to_rail_XY@100, to_ball3_23_Z@1 <-> to_rail_Z@100, to_ball3_23_YZ@1 <-> to_rail_YZ@100
101. SAR3_ba:98 — to_ball3_24_XY@1 <-> to_rail_XY@101, to_ball3_24_Z@1 <-> to_rail_Z@101, to_ball3_24_YZ@1 <-> to_rail_YZ@101
102. SAR3_ba:99 — to_ball3_25_XY@1 <-> to_rail_XY@102, to_ball3_25_Z@1 <-> to_rail_Z@102, to_ball3_25_YZ@1 <-> to_rail_YZ@102
103. SAR3_ba:100 — to_ball3_26_XY@1 <-> to_rail_XY@103, to_ball3_26_Z@1 <-> to_rail_Z@103, to_ball3_26_YZ@1 <-> to_rail_YZ@103
104. SAR3_ba:101 — to_ball3_27_XY@1 <-> to_rail_XY@104, to_ball3_27_Z@1 <-> to_rail_Z@104, to_ball3_27_YZ@1 <-> to_rail_YZ@104
105. SAR3_ba:102 — to_ball3_28_XY@1 <-> to_rail_XY@105, to_ball3_28_Z@1 <-> to_rail_Z@105, to_ball3_28_YZ@1 <-> to_rail_YZ@105
106. SAR3_ba:103 — to_ball3_29_XY@1 <-> to_rail_XY@106, to_ball3_29_Z@1 <-> to_rail_Z@106, to_ball3_29_YZ@1 <-> to_rail_YZ@106
107. SAR3_ba:104 — to_ball3_30_XY@1 <-> to_rail_XY@107, to_ball3_30_Z@1 <-> to_rail_Z@107, to_ball3_30_YZ@1 <-> to_rail_YZ@107
108. SAR3_ba:105 — to_ball3_31_XY@1 <-> to_rail_XY@108, to_ball3_31_Z@1 <-> to_rail_Z@108, to_ball3_31_YZ@1 <-> to_rail_YZ@108
109. SAR3_ba:106 — to_ball3_32_XY@1 <-> to_rail_XY@109, to_ball3_32_Z@1 <-> to_rail_Z@109, to_ball3_32_YZ@1 <-> to_rail_YZ@109
110. SAR3_ba:107 — to_ball3_33_XY@1 <-> to_rail_XY@110, to_ball3_33_Z@1 <-> to_rail_Z@110, to_ball3_33_YZ@1 <-> to_rail_YZ@110
111. SAR3_ba:108 — to_ball3_34_XY@1 <-> to_rail_XY@111, to_ball3_34_Z@1 <-> to_rail_Z@111, to_ball3_34_YZ@1 <-> to_rail_YZ@111
112. SAR3_ba:109 — to_ball3_35_XY@1 <-> to_rail_XY@112, to_ball3_35_Z@1 <-> to_rail_Z@112, to_ball3_35_YZ@1 <-> to_rail_YZ@112
113. SAR3_ba:110 — to_ball3_36_XY@1 <-> to_rail_XY@113, to_ball3_36_Z@1 <-> to_rail_Z@113, to_ball3_36_YZ@1 <-> to_rail_YZ@113
114. SAR3_ba:111 — to_ball3_37_XY@1 <-> to_rail_XY@114, to_ball3_37_Z@1 <-> to_rail_Z@114, to_ball3_37_YZ@1 <-> to_rail_YZ@114
115. SAR3_ba:112 — to_ball4_1_XY@1 <-> to_rail_XY@115, to_ball4_1_Z@1 <-> to_rail_Z@115, to_ball4_1_YZ@1 <-> to_rail_YZ@115
116. SAR3_ba:113 — to_ball4_2_XY@1 <-> to_rail_XY@116, to_ball4_2_Z@1 <-> to_rail_Z@116, to_ball4_2_YZ@1 <-> to_rail_YZ@116
117. SAR3_ba:114 — to_ball4_3_XY@1 <-> to_rail_XY@117, to_ball4_3_Z@1 <-> to_rail_Z@117, to_ball4_3_YZ@1 <-> to_rail_YZ@117
118. SAR3_ba:115 — to_ball4_4_XY@1 <-> to_rail_XY@118, to_ball4_4_Z@1 <-> to_rail_Z@118, to_ball4_4_YZ@1 <-> to_rail_YZ@118
119. SAR3_ba:116 — to_ball4_5_XY@1 <-> to_rail_XY@119, to_ball4_5_Z@1 <-> to_rail_Z@119, to_ball4_5_YZ@1 <-> to_rail_YZ@119
120. SAR3_ba:117 — to_ball4_6_XY@1 <-> to_rail_XY@120, to_ball4_6_Z@1 <-> to_rail_Z@120, to_ball4_6_YZ@1 <-> to_rail_YZ@120
121. SAR3_ba:118 — to_ball4_7_XY@1 <-> to_rail_XY@121, to_ball4_7_Z@1 <-> to_rail_Z@121, to_ball4_7_YZ@1 <-> to_rail_YZ@121
122. SAR3_ba:119 — to_ball4_8_XY@1 <-> to_rail_XY@122, to_ball4_8_Z@1 <-> to_rail_Z@122, to_ball4_8_YZ@1 <-> to_rail_YZ@122
123. SAR3_ba:120 — to_ball4_9_XY@1 <-> to_rail_XY@123, to_ball4_9_Z@1 <-> to_rail_Z@123, to_ball4_9_YZ@1 <-> to_rail_YZ@123
124. SAR3_ba:121 — to_ball4_10_XY@1 <-> to_rail_XY@124, to_ball4_10_Z@1 <-> to_rail_Z@124, to_ball4_10_YZ@1 <-> to_rail_YZ@124
125. SAR3_ba:122 — to_ball4_11_XY@1 <-> to_rail_XY@125, to_ball4_11_Z@1 <-> to_rail_Z@125, to_ball4_11_YZ@1 <-> to_rail_YZ@125
126. SAR3_ba:123 — to_ball4_12_XY@1 <-> to_rail_XY@126, to_ball4_12_Z@1 <-> to_rail_Z@126, to_ball4_12_YZ@1 <-> to_rail_YZ@126
127. SAR3_ba:124 — to_ball4_13_XY@1 <-> to_rail_XY@127, to_ball4_13_Z@1 <-> to_rail_Z@127, to_ball4_13_YZ@1 <-> to_rail_YZ@127
128. SAR3_ba:125 — to_ball4_14_XY@1 <-> to_rail_XY@128, to_ball4_14_Z@1 <-> to_rail_Z@128, to_ball4_14_YZ@1 <-> to_rail_YZ@128
129. SAR3_ba:126 — to_ball4_15_XY@1 <-> to_rail_XY@129, to_ball4_15_Z@1 <-> to_rail_Z@129, to_ball4_15_YZ@1 <-> to_rail_YZ@129
130. SAR3_ba:127 — to_ball4_16_XY@1 <-> to_rail_XY@130, to_ball4_16_Z@1 <-> to_rail_Z@130, to_ball4_16_YZ@1 <-> to_rail_YZ@130
131. SAR3_ba:128 — to_ball4_17_XY@1 <-> to_rail_XY@131, to_ball4_17_Z@1 <-> to_rail_Z@131, to_ball4_17_YZ@1 <-> to_rail_YZ@131
132. SAR3_ba:129 — to_ball4_18_XY@1 <-> to_rail_XY@132, to_ball4_18_Z@1 <-> to_rail_Z@132, to_ball4_18_YZ@1 <-> to_rail_YZ@132
133. SAR3_ba:130 — to_ball4_19_XY@1 <-> to_rail_XY@133, to_ball4_19_Z@1 <-> to_rail_Z@133, to_ball4_19_YZ@1 <-> to_rail_YZ@133
134. SAR3_ba:131 — to_ball4_20_XY@1 <-> to_rail_XY@134, to_ball4_20_Z@1 <-> to_rail_Z@134, to_ball4_20_YZ@1 <-> to_rail_YZ@134
135. SAR3_ba:132 — to_ball4_21_XY@1 <-> to_rail_XY@135, to_ball4_21_Z@1 <-> to_rail_Z@135, to_ball4_21_YZ@1 <-> to_rail_YZ@135
136. SAR3_ba:133 — to_ball4_22_XY@1 <-> to_rail_XY@136, to_ball4_22_Z@1 <-> to_rail_Z@136, to_ball4_22_YZ@1 <-> to_rail_YZ@136
137. SAR3_ba:134 — to_ball4_23_XY@1 <-> to_rail_XY@137, to_ball4_23_Z@1 <-> to_rail_Z@137, to_ball4_23_YZ@1 <-> to_rail_YZ@137
138. SAR3_ba:135 — to_ball4_24_XY@1 <-> to_rail_XY@138, to_ball4_24_Z@1 <-> to_rail_Z@138, to_ball4_24_YZ@1 <-> to_rail_YZ@138
139. SAR3_ba:136 — to_ball4_25_XY@1 <-> to_rail_XY@139, to_ball4_25_Z@1 <-> to_rail_Z@139, to_ball4_25_YZ@1 <-> to_rail_YZ@139
140. SAR3_ba:137 — to_ball4_26_XY@1 <-> to_rail_XY@140, to_ball4_26_Z@1 <-> to_rail_Z@140, to_ball4_26_YZ@1 <-> to_rail_YZ@140
141. SAR3_ba:138 — to_ball4_27_XY@1 <-> to_rail_XY@141, to_ball4_27_Z@1 <-> to_rail_Z@141, to_ball4_27_YZ@1 <-> to_rail_YZ@141
142. SAR3_ba:139 — to_ball4_28_XY@1 <-> to_rail_XY@142, to_ball4_28_Z@1 <-> to_rail_Z@142, to_ball4_28_YZ@1 <-> to_rail_YZ@142
143. SAR3_ba:140 — to_ball4_29_XY@1 <-> to_rail_XY@143, to_ball4_29_Z@1 <-> to_rail_Z@143, to_ball4_29_YZ@1 <-> to_rail_YZ@143
144. SAR3_ba:141 — to_ball4_30_XY@1 <-> to_rail_XY@144, to_ball4_30_Z@1 <-> to_rail_Z@144, to_ball4_30_YZ@1 <-> to_rail_YZ@144
145. SAR3_ba:142 — to_ball4_31_XY@1 <-> to_rail_XY@145, to_ball4_31_Z@1 <-> to_rail_Z@145, to_ball4_31_YZ@1 <-> to_rail_YZ@145
146. SAR3_ba:143 — to_ball4_32_XY@1 <-> to_rail_XY@146, to_ball4_32_Z@1 <-> to_rail_Z@146, to_ball4_32_YZ@1 <-> to_rail_YZ@146
147. SAR3_ba:144 — to_ball4_33_XY@1 <-> to_rail_XY@147, to_ball4_33_Z@1 <-> to_rail_Z@147, to_ball4_33_YZ@1 <-> to_rail_YZ@147
148. SAR3_ba:145 — to_ball4_34_XY@1 <-> to_rail_XY@148, to_ball4_34_Z@1 <-> to_rail_Z@148, to_ball4_34_YZ@1 <-> to_rail_YZ@148
149. SAR3_ba:146 — to_ball4_35_XY@1 <-> to_rail_XY@149, to_ball4_35_Z@1 <-> to_rail_Z@149, to_ball4_35_YZ@1 <-> to_rail_YZ@149
150. SAR3_ba:147 — to_ball4_36_XY@1 <-> to_rail_XY@150, to_ball4_36_Z@1 <-> to_rail_Z@150, to_ball4_36_YZ@1 <-> to_rail_YZ@150
151. SAR3_ba:148 — to_ball4_37_XY@1 <-> to_rail_XY@151, to_ball4_37_Z@1 <-> to_rail_Z@151, to_ball4_37_YZ@1 <-> to_rail_YZ@151
## Relationships (454: Mate 304, Angle 150)
- to_body_Z@1 <-> to_rail_Z@2 [Mate]: SAR340-40_r:1 ↔ SAR340-40_b:1
- to_body_YZ@1 <-> to_rail_YZ@2 [Angle] (0 deg): SAR340-40_r:1 ↔ SAR340-40_b:1
- to_body2_Z@1 <-> to_rail_Z@3 [Mate]: SAR340-40_r:1 ↔ SAR340-40_b:2
- to_body2_YZ@1 <-> to_rail_YZ@3 [Angle] (180 deg): SAR340-40_r:1 ↔ SAR340-40_b:2
- to_ball1_1_XY@1 <-> to_rail_XY@4 [Mate]: SAR340-40_r:1 ↔ SAR3_ba:1
- to_ball1_1_Z@1 <-> to_rail_Z@4 [Mate]: SAR340-40_r:1 ↔ SAR3_ba:1
- to_ball1_1_YZ@1 <-> to_rail_YZ@4 [Angle] (0 deg): SAR340-40_r:1 ↔ SAR3_ba:1
- to_ball1_2_XY@1 <-> to_rail_XY@5 [Mate]: SAR340-40_r:1 ↔ SAR3_ba:2
- to_ball1_2_Z@1 <-> to_rail_Z@5 [Mate]: SAR340-40_r:1 ↔ SAR3_ba:2
- to_ball1_2_YZ@1 <-> to_rail_YZ@5 [Angle] (0 deg): SAR340-40_r:1 ↔ SAR3_ba:2
- to_ball1_3_XY@1 <-> to_rail_XY@6 [Mate]: SAR340-40_r:1 ↔ SAR3_ba:3
- to_ball1_3_Z@1 <-> to_rail_Z@6 [Mate]: SAR340-40_r:1 ↔ SAR3_ba:3
- to_ball1_3_YZ@1 <-> to_rail_YZ@6 [Angle] (0 deg): SAR340-40_r:1 ↔ SAR3_ba:3
- to_ball1_4_XY@1 <-> to_rail_XY@7 [Mate]: SAR340-40_r:1 ↔ SAR3_ba:4
- to_ball1_4_Z@1 <-> to_rail_Z@7 [Mate]: SAR340-40_r:1 ↔ SAR3_ba:4
- to_ball1_4_YZ@1 <-> to_rail_YZ@7 [Angle] (0 deg): SAR340-40_r:1 ↔ SAR3_ba:4
- to_ball1_5_XY@1 <-> to_rail_XY@8 [Mate]: SAR340-40_r:1 ↔ SAR3_ba:5
- to_ball1_5_Z@1 <-> to_rail_Z@8 [Mate]: SAR340-40_r:1 ↔ SAR3_ba:5
- to_ball1_5_YZ@1 <-> to_rail_YZ@8 [Angle] (0 deg): SAR340-40_r:1 ↔ SAR3_ba:5
- to_ball1_6_XY@1 <-> to_rail_XY@9 [Mate]: SAR340-40_r:1 ↔ SAR3_ba:6
- to_ball1_6_Z@1 <-> to_rail_Z@9 [Mate]: SAR340-40_r:1 ↔ SAR3_ba:6
- to_ball1_6_YZ@1 <-> to_rail_YZ@9 [Angle] (0 deg): SAR340-40_r:1 ↔ SAR3_ba:6
- to_ball1_7_XY@1 <-> to_rail_XY@10 [Mate]: SAR340-40_r:1 ↔ SAR3_ba:7
- to_ball1_7_Z@1 <-> to_rail_Z@10 [Mate]: SAR340-40_r:1 ↔ SAR3_ba:7